# Autodesk Inventor assembly: リンク_ふくらはぎ_前_1
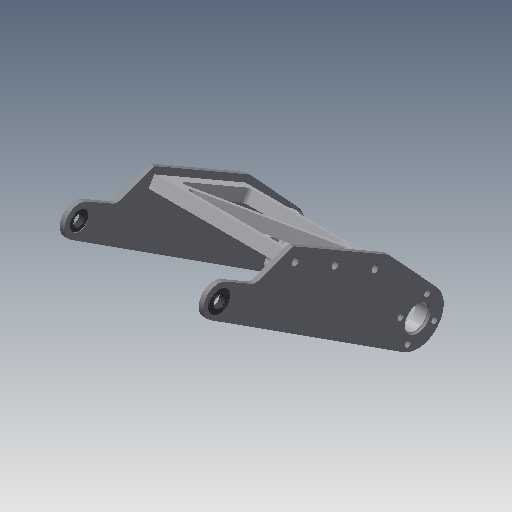
[picture p0: Inventor's stored thumbnail of the model, 512x512]
Saved by Autodesk Inventor 2017.3 (Build 213256000, 256)
## iProperties
Created: 2016-04-29
Part Number: リンク_ふくらはぎ_前_1
Document SubType Name: Assembly
Designer: hiroaki
Mass: 56.0755 g
Surface Area: 183.303 cm^2
Volume: 15.7731 cm^3
Density: 3.55513 g/cm^3
Author: hiroaki
## Documents named in this file (5)
- C:\Users\haya\Desktop\GankenKun0_5\下半身\リンク\ふくらはぎ\リンク_ふくらはぎ_前_1.iam
- C:\Users\haya\Desktop\GankenKun0_5\下半身\リンク\ふくらはぎ\リンク_ふくらはぎ_メインフレーム_1_1.ipt
- C:\Users\haya\Desktop\GankenKun0_5\既製品\NSK_RB_MF85ZZ\MF85ZZ.iam
- C:\Users\haya\Desktop\GankenKun0_5\下半身\リンク\ふくらはぎ\リンク_ふくらはぎ_サブフレーム_1_4.ipt
- C:\Users\haya\Desktop\GankenKun0_5\下半身\リンク\ふくらはぎ\リンク_ふくらはぎ_サブフレーム_1_1(予備案).ipt
## Components (7 placed, 4 different names)
1. リンク_ふくらはぎ_メインフレーム_1_1:1 — 挿入:8, 挿入:16, 挿入:20, 挿入:21, 挿入:22, 挿入:23, 挿入:24
2. リンク_ふくらはぎ_メインフレーム_1_1:2 — 挿入:7, 挿入:15, 挿入:18, 挿入:19, 挿入:25, 挿入:26, 挿入:27
3. MF85ZZ:1 [sub-assembly] — 挿入:7
4. MF85ZZ:2 [sub-assembly] — 挿入:8
5. リンク_ふくらはぎ_サブフレーム_1_4:1 — 挿入:15, 挿入:18, 挿入:19
6. リンク_ふくらはぎ_サブフレーム_1_4:2 — 挿入:16, 挿入:20, 挿入:21
7. リンク_ふくらはぎ_サブフレーム_1_1(予備案):1 — 挿入:22, 挿入:23, 挿入:24, 挿入:25, 挿入:26, 挿入:27
## Relationships (14: Insert 14)
- 挿入:7 [Insert]: リンク_ふくらはぎ_メインフレーム_1_1:2 ↔ MF85ZZ:1
- 挿入:8 [Insert]: リンク_ふくらはぎ_メインフレーム_1_1:1 ↔ MF85ZZ:2
- 挿入:15 [Insert]: リンク_ふくらはぎ_メインフレーム_1_1:2 ↔ リンク_ふくらはぎ_サブフレーム_1_4:1
- 挿入:16 [Insert]: リンク_ふくらはぎ_メインフレーム_1_1:1 ↔ リンク_ふくらはぎ_サブフレーム_1_4:2
- 挿入:18 [Insert]: リンク_ふくらはぎ_メインフレーム_1_1:2 ↔ リンク_ふくらはぎ_サブフレーム_1_4:1
- 挿入:19 [Insert]: リンク_ふくらはぎ_メインフレーム_1_1:2 ↔ リンク_ふくらはぎ_サブフレーム_1_4:1
- 挿入:20 [Insert]: リンク_ふくらはぎ_メインフレーム_1_1:1 ↔ リンク_ふくらはぎ_サブフレーム_1_4:2
- 挿入:21 [Insert]: リンク_ふくらはぎ_メインフレーム_1_1:1 ↔ リンク_ふくらはぎ_サブフレーム_1_4:2
- 挿入:22 [Insert]: リンク_ふくらはぎ_メインフレーム_1_1:1 ↔ リンク_ふくらはぎ_サブフレーム_1_1(予備案):1
- 挿入:23 [Insert]: リンク_ふくらはぎ_メインフレーム_1_1:1 ↔ リンク_ふくらはぎ_サブフレーム_1_1(予備案):1
- 挿入:24 [Insert]: リンク_ふくらはぎ_メインフレーム_1_1:1 ↔ リンク_ふくらはぎ_サブフレーム_1_1(予備案):1
- 挿入:25 [Insert]: リンク_ふくらはぎ_メインフレーム_1_1:2 ↔ リンク_ふくらはぎ_サブフレーム_1_1(予備案):1
- 挿入:26 [Insert]: リンク_ふくらはぎ_メインフレーム_1_1:2 ↔ リンク_ふくらはぎ_サブフレーム_1_1(予備案):1
- 挿入:27 [Insert]: リンク_ふくらはぎ_メインフレーム_1_1:2 ↔ リンク_ふくらはぎ_サブフレーム_1_1(予備案):1
